# Autodesk Inventor assembly: NewChassis
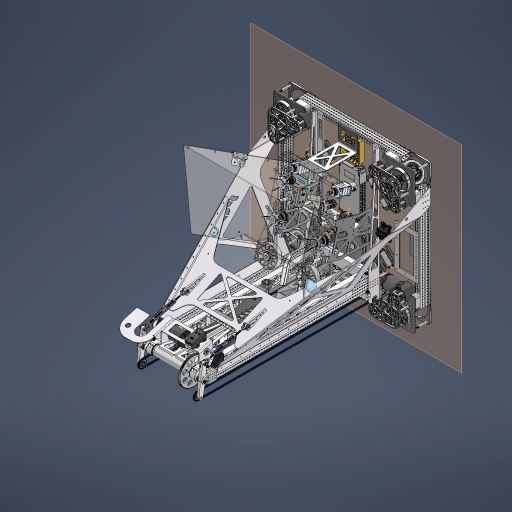
[picture p0: Inventor's stored thumbnail of the model, 512x512]
Saved by Autodesk Inventor 2024.3 (Build 283343000, 343)
## iProperties
ILogicPurgeVersion: 0.0.0.0
OnSaveVersion: 3.5.0.0
OnSaveAssembly: COREAutomationManager
Created: 2025-01-13
Part Number: NewChassis
Document SubType Name: Assembly
Designer: Marcus Tannini
Mfg Approved By: John.Thibert
Mass: 42479.6 g
Surface Area: 120890 cm^2
Volume: 18550.7 cm^3
Density: 2.28991 g/cm^3
ModelCat: Uncategorized
CN_MASS: 42.48
Author: Marcus Tannini
## Documents named in this file (46)
- \\clfs\homes\john.thibert\2025-Poseidon-Mechanical\#Poseidon 2025.iam
- \\clfs\homes\john.thibert\2025-Poseidon-Mechanical\ASSY,MK4i,Swerve_Module_INV.iam
- \\clfs\homes\john.thibert\2025-Poseidon-Mechanical\MAXTube-2x1-Holes.ipt
- \\clfs\homes\john.thibert\2025-Poseidon-Mechanical\BellyPanTop.ipt
- \\clfs\homes\john.thibert\2025-Poseidon-Mechanical\BellyPanBot.ipt
- \\clfs\homes\john.thibert\2025-Poseidon-Mechanical\BATTERY,12V.ipt
- \\clfs\homes\john.thibert\2025-Poseidon-Mechanical\CONTROLS,MAIN_BREAKER.ipt
- \\clfs\homes\john.thibert\2025-Poseidon-Mechanical\CONTROLS,MOTOR,NEO,550.ipt
- \\clfs\homes\john.thibert\2025-Poseidon-Mechanical\CONTROLS,PDH.ipt
- \\clfs\homes\john.thibert\2025-Poseidon-Mechanical\CONTROLS,PH.ipt
- \\clfs\homes\john.thibert\2025-Poseidon-Mechanical\CONTROLS,ROBO_RIO.ipt
- \\clfs\homes\john.thibert\2025-Poseidon-Mechanical\CONTROLS,SPARK_MAX.ipt
- \\clfs\homes\john.thibert\2025-Poseidon-Mechanical\CONTROLS,VRM.ipt
- \\clfs\homes\john.thibert\2025-Poseidon-Mechanical\COVER,SPARKMAX.ipt
- \\clfs\homes\john.thibert\2025-Poseidon-Mechanical\ModifiedCase(IncludesPatterning).iam
- \\clfs\homes\john.thibert\2025-Poseidon-Mechanical\PLATE,MOUNT,BATTERY,TOP.ipt
- \\clfs\homes\john.thibert\2025-Poseidon-Mechanical\SPACER,SPROCKET,IDLER,ELEVATOR.ipt
- \\clfs\homes\john.thibert\2025-Poseidon-Mechanical\PLATE,SIDE,BRACE,RIGHT,ELEVATOR.ipt
- \\clfs\homes\john.thibert\2025-Poseidon-Mechanical\PLATE,SIDE,BRACE,LEFT,ELEVATOR.ipt
- \\clfs\homes\john.thibert\2025-Poseidon-Mechanical\PLATE,TURNBUCKLE,TENSIONER,CHAIN.ipt
- \\clfs\homes\john.thibert\2025-Poseidon-Mechanical\PLATE,BRACE,HORISONTAL,TOP,ELEVATOR.ipt
- \\clfs\homes\john.thibert\2025-Poseidon-Mechanical\TURNBUCKLE,0.25IN_CLEVIS.iam
- \\clfs\homes\john.thibert\2025-Poseidon-Mechanical\STAGE1,ELEVATOR.iam
- \\clfs\homes\john.thibert\2025-Poseidon-Mechanical\ASSY,MAIN,ELEVATOR.iam
- \\clfs\homes\john.thibert\2025-Poseidon-Mechanical\ANGLE,MOUNT,ELEVATOR.ipt
- \\clfs\homes\john.thibert\2025-Poseidon-Mechanical\ANGLE,MOUNT,ELEVATOR,MIRR.ipt
- \\clfs\homes\john.thibert\2025-Poseidon-Mechanical\FABRIC,BUMPERS.ipt
- \\clfs\homes\john.thibert\2025-Poseidon-Mechanical\9293K119_Constant-Force Spring.ipt
- \\clfs\homes\john.thibert\2025-Poseidon-Mechanical\MOUNT,SPRING,ELEVATOR.ipt
- \\clfs\homes\john.thibert\2025-Poseidon-Mechanical\MOUNT,SPRING,ELEVATOR,MIRR.ipt
- \\clfs\homes\john.thibert\2025-Poseidon-Mechanical\SPACER,HEX,0.125IN.ipt
- \\clfs\homes\john.thibert\2025-Poseidon-Mechanical\ARM.iam
- \\clfs\homes\john.thibert\2025-Poseidon-Mechanical\DRIVETRAIN,ELEVATOR.iam
- \\clfs\homes\john.thibert\2025-Poseidon-Mechanical\hopper_assy.iam
- \\clfs\homes\john.thibert\2025-Poseidon-Mechanical\feeder_front_support.ipt
- \\clfs\homes\john.thibert\2025-Poseidon-Mechanical\coral_end_stop.ipt
- \\clfs\homes\john.thibert\2025-Poseidon-Mechanical\coral_end_stop_MIR.ipt
- \\clfs\homes\john.thibert\2025-Poseidon-Mechanical\hopper_backboard.ipt
- \\clfs\homes\john.thibert\2025-Poseidon-Mechanical\Part Studio 1 - Support 1.ipt
- \\clfs\homes\john.thibert\2025-Poseidon-Mechanical\Part Studio 1 - Support 2.ipt
- \\clfs\homes\john.thibert\2025-Poseidon-Mechanical\SDS COLSON.ipt
- \\clfs\homes\john.thibert\2025-Poseidon-Mechanical\SDS LOWERING SPACER.ipt
- \\clfs\homes\john.thibert\2025-Poseidon-Mechanical\#Poseidon 2025\Design Accelerator\Spur Gear21.ipt
- \\clfs\homes\john.thibert\2025-Poseidon-Mechanical\#Poseidon 2025\Design Accelerator\Spur Gear11.ipt
- \\clfs\homes\john.thibert\2025-Poseidon-Mechanical\PLATE,SUPPORT,STOP,ARM.ipt
- \\clfs\homes\john.thibert\2025-Poseidon-Mechanical\PLATE,BRACKET,CABLE_CHAIN.ipt
## Components (81 placed, 47 different names)
1. FABRIC,BUMPERS.ipt:1 — Flush:323, Mate:335, Mate:336
2. Spur Gear1:1 — Mate:708, Mate:709, Flush:325, Rotation:1, Mate:712
3. Spur Gear2:1 — Mate:710, Flush:325, Rotation:1
4. ARM:1 [sub-assembly] — Angle:1, Mate:708, Mate:709, Mate:712, ARM-ANGLE
5. PLATE,BRACKET,CABLE_CHAIN:1 — Flush:326, Mate:722, Mate:723
6. BellyPanBot.ipt:1 — Mate:66, Mate:353, Mate:354
7. BellyPanTop.ipt:1 — Mate:62, Mate:63, Mate:65, Mate:70, Mate:71, Mate:82, Mate:84, Insert:7, Insert:8, Insert:9, Insert:10, Insert:11, Insert:12, Insert:13, Insert:14, Insert:15, Insert:16, Insert:17, Insert:18, Insert:19, Insert:20, Insert:21, Insert:22, Mate:111, Mate:113, Mate:114, Mate:116, Mate:117, Mate:118, Mate:119, Mate:121, Mate:122, Mate:123, Mate:124, Mate:125, Mate:126, Mate:127, Mate:130, Insert:23, Insert:24, Mate:308, Mate:349, Mate:350, Mate:659, Mate:660, Mate:661
8. MAXTube-2x1-Holes.ipt:1 — Mate:3, Mate:4, Mate:115, Mate:272, Mate:687, Mate:692, Mate:696
9. MAXTube-2x1-Holes.ipt:2 — Mate:6, Mate:7, Mate:9, Mate:10, Mate:62, Mate:309, Mate:310
10. MAXTube-2x1-Holes.ipt:3 — Mate:19, Mate:20, Mate:66, Mate:114, Mate:312, Mate:313, Mate:336, Mate:691, Mate:703
11. MAXTube-2x1-Holes.ipt:4 — Mate:12, Mate:13, Mate:16, Mate:17, Mate:29, Mate:63, Mate:271, Mate:353, Mate:354, Mate:678
12. BATTERY,12V.ipt:1 — Mate:356
13. CONTROLS,MAIN_BREAKER.ipt:1 — Mate:82, Mate:111, Mate:116
14. CONTROLS,MOTOR,NEO,550.ipt:1
15. CONTROLS,PDH.ipt:1 — Mate:113, Mate:117, Mate:118, Mate:119
16. CONTROLS,PH.ipt:1 — Insert:23, Insert:24
17. CONTROLS,ROBO_RIO.ipt:1 — Mate:124, Mate:125, Mate:126
18. CONTROLS,SPARK_MAX.ipt:1 — Mate:84, Mate:85, Mate:86, Mate:87
19. CONTROLS,VRM.ipt:1 — Mate:121, Mate:122, Mate:123
20. ModifiedCase(IncludesPatterning).iam:1 [sub-assembly] — Mate:130
21. PLATE,MOUNT,BATTERY,TOP.ipt:1 — Mate:127, Mate:349, Mate:350, Mate:356
22. COVER,SPARKMAX:9 — Mate:724
23. CONTROLS,SPARK_MAX:9 — Mate:655
24. PLATE,SUPPORT,STOP,ARM:1 — Mate:720, Mate:721
25. ASSY,MAIN,ELEVATOR.iam:1 [sub-assembly] — Mate:161, Mate:162, Flush:19, Mate:297, STAGE1 UPPER LIMIT, STAGE1 MAX, Mate:311, Mate:314, Mate:315, Mate:363, Mate:362, Mate:366, Mate:367, Mate:368, Mate:369
26. DRIVETRAIN,ELEVATOR:1 [sub-assembly]
27. STAGE1,ELEVATOR.iam:1 [sub-assembly] — Flush:19, Mate:297, STAGE1 LOWER LIMIT, STAGE1 UPPER LIMIT, STAGE1 DRIVE, STAGE1 MAX, Angle:1, Mate:655, Mate:710, Mate:720, Mate:721, Flush:326, Mate:722, Mate:723, Mate:724, ARM-ANGLE
28. TURNBUCKLE,0.25IN_CLEVIS.iam:1 [sub-assembly]
29. TURNBUCKLE,0.25IN_CLEVIS.iam:2 [sub-assembly] — Mate:707
30. 9293K119_Constant-Force Spring:1 — Mate:364, Mate:365
31. 9293K119_Constant-Force Spring:2 — Mate:370, Mate:371
32. ANGLE,MOUNT,ELEVATOR,MIRR.ipt:1 — Mate:308, Mate:309, Mate:310, Mate:311, Mate:312, Mate:313, Mate:314, Mate:315, Mate:656, Mate:657, Mate:658
33. ANGLE,MOUNT,ELEVATOR.ipt:1 — Mate:65, Mate:70, Mate:71, Mate:161, Mate:162, STAGE1 LOWER LIMIT, STAGE1 DRIVE
34. MOUNT,SPRING,ELEVATOR,MIRR:1 — Mate:367, Mate:368, Mate:369, Mate:370, Mate:371
35. MOUNT,SPRING,ELEVATOR:1 — Mate:363, Mate:362, Mate:364, Mate:365, Mate:366
36. PLATE,BRACE,HORISONTAL,TOP,ELEVATOR.ipt:1 — Mate:285, Mate:286, Mate:289, Mate:290, Mate:291, Mate:295, Mate:296, Mate:668, Mate:669, Mate:670
37. PLATE,SIDE,BRACE,LEFT,ELEVATOR.ipt:1 — Mate:271, Mate:289, Mate:290, Mate:291, Mate:335
38. PLATE,SIDE,BRACE,RIGHT,ELEVATOR.ipt:1 — Mate:272
39. PLATE,TURNBUCKLE,TENSIONER,CHAIN.ipt:1 — Mate:285, Mate:296
40. PLATE,TURNBUCKLE,TENSIONER,CHAIN.ipt:2 — Mate:286, Mate:295, Mate:707
41. SPACER,HEX,0.125IN:1
42. SPACER,SPROCKET,IDLER,ELEVATOR.ipt:1
43. SPACER,SPROCKET,IDLER,ELEVATOR.ipt:2
44. SDS COLSON:1 — Insert:52
45. SDS COLSON:2 — Insert:49
46. SDS COLSON:3 — Insert:50
47. SDS COLSON:4 — Insert:51
48. SDS LOWERING SPACER:1 — Mate:677, Mate:678, Mate:679, Mate:680
49. SDS LOWERING SPACER:2 — Mate:681, Mate:682, Mate:683
50. SDS LOWERING SPACER:3 — Mate:688, Mate:689, Mate:690
51. SDS LOWERING SPACER:4 — Mate:684, Mate:685, Mate:686, Mate:687
52. SDS LOWERING SPACER:5 — Mate:693, Mate:694, Mate:695, Mate:696
53. SDS LOWERING SPACER:6 — Mate:697, Mate:698, Mate:699
54. SDS LOWERING SPACER:7 — Mate:700, Mate:701, Mate:702, Mate:703
55. SDS LOWERING SPACER:8 — Mate:704, Mate:705, Mate:706
56. ASSY,MK4i,Swerve_Module_INV.iam:1 [sub-assembly] — Insert:50, Mate:691, Mate:692, Mate:693, Mate:694, Mate:695, Mate:697, Mate:698, Mate:699
57. ASSY,MK4i,Swerve_Module_INV.iam:2 [sub-assembly] — Mate:3, Mate:4, Mate:6, Mate:7, Insert:51, Mate:684, Mate:685, Mate:686, Mate:688, Mate:689, Mate:690
58. ASSY,MK4i,Swerve_Module_INV.iam:3 [sub-assembly] — Mate:9, Mate:10, Mate:12, Mate:13, Insert:52, Mate:677, Mate:679, Mate:680, Mate:681, Mate:682, Mate:683
59. ASSY,MK4i,Swerve_Module_INV.iam:4 [sub-assembly] — Mate:16, Mate:17, Mate:19, Mate:20, Mate:67, Insert:49, Mate:700, Mate:701, Mate:702, Mate:704, Mate:705, Mate:706
60. CONTROLS,SPARK_MAX.ipt:2
61. CONTROLS,SPARK_MAX.ipt:3
62. CONTROLS,SPARK_MAX.ipt:4
63. CONTROLS,SPARK_MAX.ipt:5
64. CONTROLS,SPARK_MAX.ipt:6
65. CONTROLS,SPARK_MAX.ipt:7
66. CONTROLS,SPARK_MAX.ipt:8
67. COVER,SPARKMAX.ipt:1 — Mate:85, Mate:86, Mate:87, Insert:7, Insert:8
68. COVER,SPARKMAX.ipt:2 — Insert:9, Insert:10
69. COVER,SPARKMAX.ipt:3 — Insert:11, Insert:12
70. COVER,SPARKMAX.ipt:4 — Insert:13, Insert:14
71. COVER,SPARKMAX.ipt:5 — Insert:17, Insert:18
72. COVER,SPARKMAX.ipt:6 — Insert:15, Insert:16
73. COVER,SPARKMAX.ipt:7 — Insert:21, Insert:22
74. COVER,SPARKMAX.ipt:8 — Insert:19, Insert:20
75. hopper_assy:1 [sub-assembly] — Mate:656, Mate:657, Mate:658, Mate:671, Mate:672, Mate:673, Mate:674, Mate:675, Mate:676
76. feeder_front_support:1 — Mate:659, Mate:660, Mate:661, Mate:662, Mate:663, Mate:664, Mate:665, Mate:666, Mate:667
77. coral_end_stop:1 — Mate:665, Mate:666, Mate:667
78. coral_end_stop_MIR:1 — Mate:662, Mate:663, Mate:664
79. hopper_backboard:1 — Mate:668, Mate:669, Mate:670
80. Part Studio 1 - Support 1:1 — Mate:674, Mate:675, Mate:676
81. Part Studio 1 - Support 2:1 — Mate:671, Mate:672, Mate:673
## Relationships (229: Mate 193, Insert 26, Flush 7, Angle 2, RelateRotation 1)
- Mate:3: MAXTube-2x1-Holes.ipt:1 ↔ ASSY,MK4i,Swerve_Module_INV.iam:2
- Mate:4: MAXTube-2x1-Holes.ipt:1 ↔ ASSY,MK4i,Swerve_Module_INV.iam:2
- Mate:6: MAXTube-2x1-Holes.ipt:2 ↔ ASSY,MK4i,Swerve_Module_INV.iam:2
- Mate:7: MAXTube-2x1-Holes.ipt:2 ↔ ASSY,MK4i,Swerve_Module_INV.iam:2
- Mate:9: MAXTube-2x1-Holes.ipt:2 ↔ ASSY,MK4i,Swerve_Module_INV.iam:3
- Mate:10: MAXTube-2x1-Holes.ipt:2 ↔ ASSY,MK4i,Swerve_Module_INV.iam:3
- Mate:12: MAXTube-2x1-Holes.ipt:4 ↔ ASSY,MK4i,Swerve_Module_INV.iam:3
- Mate:13: MAXTube-2x1-Holes.ipt:4 ↔ ASSY,MK4i,Swerve_Module_INV.iam:3
- Mate:16: MAXTube-2x1-Holes.ipt:4 ↔ ASSY,MK4i,Swerve_Module_INV.iam:4
- Mate:17: MAXTube-2x1-Holes.ipt:4 ↔ ASSY,MK4i,Swerve_Module_INV.iam:4
- Mate:19: MAXTube-2x1-Holes.ipt:3 ↔ ASSY,MK4i,Swerve_Module_INV.iam:4
- Mate:20: MAXTube-2x1-Holes.ipt:3 ↔ ASSY,MK4i,Swerve_Module_INV.iam:4
- Mate:29 (-6.35 mm): MAXTube-2x1-Holes.ipt:4
- Mate:62: BellyPanTop.ipt:1 ↔ MAXTube-2x1-Holes.ipt:2
- Mate:63: BellyPanTop.ipt:1 ↔ MAXTube-2x1-Holes.ipt:4
- Mate:65: BellyPanTop.ipt:1 ↔ ANGLE,MOUNT,ELEVATOR.ipt:1
- Mate:66: BellyPanBot.ipt:1 ↔ MAXTube-2x1-Holes.ipt:3
- Mate:67 (35.56 mm): ASSY,MK4i,Swerve_Module_INV.iam:4
- Mate:70: BellyPanTop.ipt:1 ↔ ANGLE,MOUNT,ELEVATOR.ipt:1
- Mate:71: BellyPanTop.ipt:1 ↔ ANGLE,MOUNT,ELEVATOR.ipt:1
- Mate:82: BellyPanTop.ipt:1 ↔ CONTROLS,MAIN_BREAKER.ipt:1
- Mate:84: BellyPanTop.ipt:1 ↔ CONTROLS,SPARK_MAX.ipt:1
- Mate:85: CONTROLS,SPARK_MAX.ipt:1 ↔ COVER,SPARKMAX.ipt:1
- Mate:86: CONTROLS,SPARK_MAX.ipt:1 ↔ COVER,SPARKMAX.ipt:1
- Mate:87: CONTROLS,SPARK_MAX.ipt:1 ↔ COVER,SPARKMAX.ipt:1
- Insert:7: BellyPanTop.ipt:1 ↔ COVER,SPARKMAX.ipt:1
- Insert:8: BellyPanTop.ipt:1 ↔ COVER,SPARKMAX.ipt:1
- [Mate]: CONTROLS,SPARK_MAX.ipt:2 ↔ COVER,SPARKMAX.ipt:2
- [Mate]: CONTROLS,SPARK_MAX.ipt:2 ↔ COVER,SPARKMAX.ipt:2
- [Mate]: CONTROLS,SPARK_MAX.ipt:2 ↔ COVER,SPARKMAX.ipt:2
- [Mate]: CONTROLS,SPARK_MAX.ipt:3 ↔ COVER,SPARKMAX.ipt:3
- [Mate]: CONTROLS,SPARK_MAX.ipt:3 ↔ COVER,SPARKMAX.ipt:3
- [Mate]: CONTROLS,SPARK_MAX.ipt:3 ↔ COVER,SPARKMAX.ipt:3
- [Mate]: CONTROLS,SPARK_MAX.ipt:4 ↔ COVER,SPARKMAX.ipt:4
- [Mate]: CONTROLS,SPARK_MAX.ipt:4 ↔ COVER,SPARKMAX.ipt:4
- [Mate]: CONTROLS,SPARK_MAX.ipt:4 ↔ COVER,SPARKMAX.ipt:4
- [Mate]: CONTROLS,SPARK_MAX.ipt:5 ↔ COVER,SPARKMAX.ipt:5
- [Mate]: CONTROLS,SPARK_MAX.ipt:5 ↔ COVER,SPARKMAX.ipt:5
- [Mate]: CONTROLS,SPARK_MAX.ipt:5 ↔ COVER,SPARKMAX.ipt:5
- [Mate]: CONTROLS,SPARK_MAX.ipt:6 ↔ COVER,SPARKMAX.ipt:6
- [Mate]: CONTROLS,SPARK_MAX.ipt:6 ↔ COVER,SPARKMAX.ipt:6
- [Mate]: CONTROLS,SPARK_MAX.ipt:6 ↔ COVER,SPARKMAX.ipt:6
- [Mate]: CONTROLS,SPARK_MAX.ipt:7 ↔ COVER,SPARKMAX.ipt:7
- [Mate]: CONTROLS,SPARK_MAX.ipt:7 ↔ COVER,SPARKMAX.ipt:7
- [Mate]: CONTROLS,SPARK_MAX.ipt:7 ↔ COVER,SPARKMAX.ipt:7
- [Mate]: CONTROLS,SPARK_MAX.ipt:8 ↔ COVER,SPARKMAX.ipt:8
- [Mate]: CONTROLS,SPARK_MAX.ipt:8 ↔ COVER,SPARKMAX.ipt:8
- [Mate]: CONTROLS,SPARK_MAX.ipt:8 ↔ COVER,SPARKMAX.ipt:8
- Insert:9: BellyPanTop.ipt:1 ↔ COVER,SPARKMAX.ipt:2
- Insert:10: BellyPanTop.ipt:1 ↔ COVER,SPARKMAX.ipt:2
- Insert:11: BellyPanTop.ipt:1 ↔ COVER,SPARKMAX.ipt:3
- Insert:12: BellyPanTop.ipt:1 ↔ COVER,SPARKMAX.ipt:3
- Insert:13: BellyPanTop.ipt:1 ↔ COVER,SPARKMAX.ipt:4
- Insert:14: BellyPanTop.ipt:1 ↔ COVER,SPARKMAX.ipt:4
- Insert:15: BellyPanTop.ipt:1 ↔ COVER,SPARKMAX.ipt:6
- Insert:16: BellyPanTop.ipt:1 ↔ COVER,SPARKMAX.ipt:6
- Insert:17: BellyPanTop.ipt:1 ↔ COVER,SPARKMAX.ipt:5
- Insert:18: BellyPanTop.ipt:1 ↔ COVER,SPARKMAX.ipt:5
- Insert:19: BellyPanTop.ipt:1 ↔ COVER,SPARKMAX.ipt:8
- Insert:20: BellyPanTop.ipt:1 ↔ COVER,SPARKMAX.ipt:8
- Insert:21: BellyPanTop.ipt:1 ↔ COVER,SPARKMAX.ipt:7
- Insert:22: BellyPanTop.ipt:1 ↔ COVER,SPARKMAX.ipt:7
- Mate:111: BellyPanTop.ipt:1 ↔ CONTROLS,MAIN_BREAKER.ipt:1
- Mate:113: BellyPanTop.ipt:1 ↔ CONTROLS,PDH.ipt:1
- Mate:114: BellyPanTop.ipt:1 ↔ MAXTube-2x1-Holes.ipt:3
- Mate:115 (-374.65 mm): MAXTube-2x1-Holes.ipt:1
- Mate:116 (0.254 mm): BellyPanTop.ipt:1 ↔ CONTROLS,MAIN_BREAKER.ipt:1
- Mate:117: BellyPanTop.ipt:1 ↔ CONTROLS,PDH.ipt:1
- Mate:118: BellyPanTop.ipt:1 ↔ CONTROLS,PDH.ipt:1
- Mate:119: BellyPanTop.ipt:1 ↔ CONTROLS,PDH.ipt:1
- Mate:121: BellyPanTop.ipt:1 ↔ CONTROLS,VRM.ipt:1
- Mate:122: BellyPanTop.ipt:1 ↔ CONTROLS,VRM.ipt:1
- Mate:123: BellyPanTop.ipt:1 ↔ CONTROLS,VRM.ipt:1
- Mate:124: BellyPanTop.ipt:1 ↔ CONTROLS,ROBO_RIO.ipt:1
- Mate:125: BellyPanTop.ipt:1 ↔ CONTROLS,ROBO_RIO.ipt:1
- Mate:126: BellyPanTop.ipt:1 ↔ CONTROLS,ROBO_RIO.ipt:1
- Mate:127: BellyPanTop.ipt:1 ↔ PLATE,MOUNT,BATTERY,TOP.ipt:1
- Mate:130: BellyPanTop.ipt:1 ↔ ModifiedCase(IncludesPatterning).iam:1
- Insert:23: BellyPanTop.ipt:1 ↔ CONTROLS,PH.ipt:1
- Insert:24: BellyPanTop.ipt:1 ↔ CONTROLS,PH.ipt:1
- Mate:161: ASSY,MAIN,ELEVATOR.iam:1 ↔ ANGLE,MOUNT,ELEVATOR.ipt:1
- Mate:162: ASSY,MAIN,ELEVATOR.iam:1 ↔ ANGLE,MOUNT,ELEVATOR.ipt:1
- [Mate]: ASSY,MAIN,ELEVATOR.iam:1 ↔ ANGLE,MOUNT,ELEVATOR.ipt:1
- [Insert]: ASSY,MAIN,ELEVATOR.iam:1 ↔ SPACER,SPROCKET,IDLER,ELEVATOR.ipt:1
- [Insert]: ASSY,MAIN,ELEVATOR.iam:1 ↔ SPACER,SPROCKET,IDLER,ELEVATOR.ipt:1
- [Flush]: ASSY,MAIN,ELEVATOR.iam:1 ↔ DRIVETRAIN,ELEVATOR:1
- [Insert]: ASSY,MAIN,ELEVATOR.iam:1 ↔ SPACER,SPROCKET,IDLER,ELEVATOR.ipt:2
- [Insert]: ASSY,MAIN,ELEVATOR.iam:1 ↔ SPACER,SPROCKET,IDLER,ELEVATOR.ipt:2
- [Mate]: BellyPanTop.ipt:1 ↔ DRIVETRAIN,ELEVATOR:1
- [Mate]: DRIVETRAIN,ELEVATOR:1 ↔ ANGLE,MOUNT,ELEVATOR.ipt:1
- [Flush]: ASSY,MAIN,ELEVATOR.iam:1 ↔ DRIVETRAIN,ELEVATOR:1
- [Mate]: ASSY,MAIN,ELEVATOR.iam:1 ↔ PLATE,SIDE,BRACE,LEFT,ELEVATOR.ipt:1
- [Mate]: ASSY,MAIN,ELEVATOR.iam:1 ↔ PLATE,SIDE,BRACE,LEFT,ELEVATOR.ipt:1
- [Mate]: ASSY,MAIN,ELEVATOR.iam:1 ↔ DRIVETRAIN,ELEVATOR:1
- [Mate]: ASSY,MAIN,ELEVATOR.iam:1 ↔ PLATE,SIDE,BRACE,LEFT,ELEVATOR.ipt:1
- [Mate]: ASSY,MAIN,ELEVATOR.iam:1 ↔ PLATE,SIDE,BRACE,RIGHT,ELEVATOR.ipt:1
- [Mate]: ASSY,MAIN,ELEVATOR.iam:1 ↔ PLATE,SIDE,BRACE,RIGHT,ELEVATOR.ipt:1
- [Mate]: ASSY,MAIN,ELEVATOR.iam:1 ↔ PLATE,SIDE,BRACE,RIGHT,ELEVATOR.ipt:1
- Mate:271: MAXTube-2x1-Holes.ipt:4 ↔ PLATE,SIDE,BRACE,LEFT,ELEVATOR.ipt:1
- Mate:272: MAXTube-2x1-Holes.ipt:1 ↔ PLATE,SIDE,BRACE,RIGHT,ELEVATOR.ipt:1
- [Mate]: ASSY,MAIN,ELEVATOR.iam:1 ↔ TURNBUCKLE,0.25IN_CLEVIS.iam:1
- [Mate]: ASSY,MAIN,ELEVATOR.iam:1 ↔ TURNBUCKLE,0.25IN_CLEVIS.iam:1
- [Mate]: ASSY,MAIN,ELEVATOR.iam:1 ↔ TURNBUCKLE,0.25IN_CLEVIS.iam:2
- [Mate]: ASSY,MAIN,ELEVATOR.iam:1 ↔ TURNBUCKLE,0.25IN_CLEVIS.iam:2
- Mate:285: PLATE,BRACE,HORISONTAL,TOP,ELEVATOR.ipt:1 ↔ PLATE,TURNBUCKLE,TENSIONER,CHAIN.ipt:1
- Mate:286: PLATE,BRACE,HORISONTAL,TOP,ELEVATOR.ipt:1 ↔ PLATE,TURNBUCKLE,TENSIONER,CHAIN.ipt:2
- Mate:289: PLATE,BRACE,HORISONTAL,TOP,ELEVATOR.ipt:1 ↔ PLATE,SIDE,BRACE,LEFT,ELEVATOR.ipt:1
- Mate:290: PLATE,BRACE,HORISONTAL,TOP,ELEVATOR.ipt:1 ↔ PLATE,SIDE,BRACE,LEFT,ELEVATOR.ipt:1
- Mate:291: PLATE,BRACE,HORISONTAL,TOP,ELEVATOR.ipt:1 ↔ PLATE,SIDE,BRACE,LEFT,ELEVATOR.ipt:1
- [Mate]: ASSY,MAIN,ELEVATOR.iam:1 ↔ DRIVETRAIN,ELEVATOR:1
- Mate:295: PLATE,BRACE,HORISONTAL,TOP,ELEVATOR.ipt:1 ↔ PLATE,TURNBUCKLE,TENSIONER,CHAIN.ipt:2
- Mate:296: PLATE,BRACE,HORISONTAL,TOP,ELEVATOR.ipt:1 ↔ PLATE,TURNBUCKLE,TENSIONER,CHAIN.ipt:1
- Flush:19: ASSY,MAIN,ELEVATOR.iam:1 ↔ STAGE1,ELEVATOR.iam:1
- Mate:297: ASSY,MAIN,ELEVATOR.iam:1 ↔ STAGE1,ELEVATOR.iam:1
- STAGE1 LOWER LIMIT [Mate]: STAGE1,ELEVATOR.iam:1 ↔ ANGLE,MOUNT,ELEVATOR.ipt:1
- STAGE1 UPPER LIMIT [Mate]: ASSY,MAIN,ELEVATOR.iam:1 ↔ STAGE1,ELEVATOR.iam:1
- STAGE1 DRIVE [Mate]: STAGE1,ELEVATOR.iam:1 ↔ ANGLE,MOUNT,ELEVATOR.ipt:1
- STAGE1 MAX [Mate] (3.175 mm): ASSY,MAIN,ELEVATOR.iam:1 ↔ STAGE1,ELEVATOR.iam:1
- Mate:308: BellyPanTop.ipt:1 ↔ ANGLE,MOUNT,ELEVATOR,MIRR.ipt:1
- Mate:309: MAXTube-2x1-Holes.ipt:2 ↔ ANGLE,MOUNT,ELEVATOR,MIRR.ipt:1
- Mate:310: MAXTube-2x1-Holes.ipt:2 ↔ ANGLE,MOUNT,ELEVATOR,MIRR.ipt:1
- Mate:311: ASSY,MAIN,ELEVATOR.iam:1 ↔ ANGLE,MOUNT,ELEVATOR,MIRR.ipt:1
- Mate:312: MAXTube-2x1-Holes.ipt:3 ↔ ANGLE,MOUNT,ELEVATOR,MIRR.ipt:1
- Mate:313: MAXTube-2x1-Holes.ipt:3 ↔ ANGLE,MOUNT,ELEVATOR,MIRR.ipt:1
- Mate:314: ASSY,MAIN,ELEVATOR.iam:1 ↔ ANGLE,MOUNT,ELEVATOR,MIRR.ipt:1
- Mate:315: ASSY,MAIN,ELEVATOR.iam:1 ↔ ANGLE,MOUNT,ELEVATOR,MIRR.ipt:1
- Flush:323 (146.05 mm): FABRIC,BUMPERS.ipt:1
- Mate:335 (3.175 mm): FABRIC,BUMPERS.ipt:1 ↔ PLATE,SIDE,BRACE,LEFT,ELEVATOR.ipt:1
- Mate:336 (6.35 mm): FABRIC,BUMPERS.ipt:1 ↔ MAXTube-2x1-Holes.ipt:3
- Mate:349: BellyPanTop.ipt:1 ↔ PLATE,MOUNT,BATTERY,TOP.ipt:1
- Mate:350: BellyPanTop.ipt:1 ↔ PLATE,MOUNT,BATTERY,TOP.ipt:1
- Mate:353: BellyPanBot.ipt:1 ↔ MAXTube-2x1-Holes.ipt:4
- Mate:354: BellyPanBot.ipt:1 ↔ MAXTube-2x1-Holes.ipt:4
- Mate:356 (19.05 mm): BATTERY,12V.ipt:1 ↔ PLATE,MOUNT,BATTERY,TOP.ipt:1
- Mate:363: ASSY,MAIN,ELEVATOR.iam:1 ↔ MOUNT,SPRING,ELEVATOR:1
- Mate:362: ASSY,MAIN,ELEVATOR.iam:1 ↔ MOUNT,SPRING,ELEVATOR:1
- Mate:364: 9293K119_Constant-Force Spring:1 ↔ MOUNT,SPRING,ELEVATOR:1
- Mate:365 (1.5875 mm): 9293K119_Constant-Force Spring:1 ↔ MOUNT,SPRING,ELEVATOR:1
- Mate:366: ASSY,MAIN,ELEVATOR.iam:1 ↔ MOUNT,SPRING,ELEVATOR:1
- Mate:367: ASSY,MAIN,ELEVATOR.iam:1 ↔ MOUNT,SPRING,ELEVATOR,MIRR:1
- Mate:368: ASSY,MAIN,ELEVATOR.iam:1 ↔ MOUNT,SPRING,ELEVATOR,MIRR:1
- Mate:369: ASSY,MAIN,ELEVATOR.iam:1 ↔ MOUNT,SPRING,ELEVATOR,MIRR:1
- Mate:370: 9293K119_Constant-Force Spring:2 ↔ MOUNT,SPRING,ELEVATOR,MIRR:1
- Mate:371 (1.5875 mm): 9293K119_Constant-Force Spring:2 ↔ MOUNT,SPRING,ELEVATOR,MIRR:1
- [Mate] (0.254 mm): ASSY,MAIN,ELEVATOR.iam:1 ↔ DRIVETRAIN,ELEVATOR:1
- [Mate]: ASSY,MAIN,ELEVATOR.iam:1 ↔ DRIVETRAIN,ELEVATOR:1
- [Mate]: DRIVETRAIN,ELEVATOR:1 ↔ SPACER,HEX,0.125IN:1
- [Mate]: DRIVETRAIN,ELEVATOR:1 ↔ SPACER,HEX,0.125IN:1
- [Mate]: ARM:1 ↔ STAGE1,ELEVATOR.iam:1
- [Mate]: ARM:1 ↔ STAGE1,ELEVATOR.iam:1
- [Mate]: MAXTube-2x1-Holes.ipt:2 ↔ DRIVETRAIN,ELEVATOR:1
- [Mate]: MAXTube-2x1-Holes.ipt:2 ↔ DRIVETRAIN,ELEVATOR:1
- [Mate]: ARM:1 ↔ STAGE1,ELEVATOR.iam:1
- [Mate]: ARM:1 ↔ STAGE1,ELEVATOR.iam:1
- Angle:1 (0 deg): ARM:1 ↔ STAGE1,ELEVATOR.iam:1
- [Mate]: COVER,SPARKMAX:9 ↔ CONTROLS,SPARK_MAX:9
- [Mate]: COVER,SPARKMAX:9 ↔ CONTROLS,SPARK_MAX:9
- [Mate]: COVER,SPARKMAX:9 ↔ CONTROLS,SPARK_MAX:9
- Mate:655: CONTROLS,SPARK_MAX:9 ↔ STAGE1,ELEVATOR.iam:1
- Mate:656: ANGLE,MOUNT,ELEVATOR,MIRR.ipt:1 ↔ hopper_assy:1
- Mate:657: ANGLE,MOUNT,ELEVATOR,MIRR.ipt:1 ↔ hopper_assy:1
- Mate:658: ANGLE,MOUNT,ELEVATOR,MIRR.ipt:1 ↔ hopper_assy:1
- Mate:659: BellyPanTop.ipt:1 ↔ feeder_front_support:1
- Mate:660: BellyPanTop.ipt:1 ↔ feeder_front_support:1
- Mate:661: BellyPanTop.ipt:1 ↔ feeder_front_support:1
- Mate:662: feeder_front_support:1 ↔ coral_end_stop_MIR:1
- Mate:663: feeder_front_support:1 ↔ coral_end_stop_MIR:1
- Mate:664: feeder_front_support:1 ↔ coral_end_stop_MIR:1
- Mate:665: feeder_front_support:1 ↔ coral_end_stop:1
- Mate:666: feeder_front_support:1 ↔ coral_end_stop:1
- Mate:667: feeder_front_support:1 ↔ coral_end_stop:1
- Mate:668: PLATE,BRACE,HORISONTAL,TOP,ELEVATOR.ipt:1 ↔ hopper_backboard:1
- Mate:669: PLATE,BRACE,HORISONTAL,TOP,ELEVATOR.ipt:1 ↔ hopper_backboard:1
- Mate:670: PLATE,BRACE,HORISONTAL,TOP,ELEVATOR.ipt:1 ↔ hopper_backboard:1
- Mate:671: hopper_assy:1 ↔ Part Studio 1 - Support 2:1
- Mate:672: hopper_assy:1 ↔ Part Studio 1 - Support 2:1
- Mate:673: hopper_assy:1 ↔ Part Studio 1 - Support 2:1
- Mate:674: hopper_assy:1 ↔ Part Studio 1 - Support 1:1
- Mate:675: hopper_assy:1 ↔ Part Studio 1 - Support 1:1
- Mate:676: hopper_assy:1 ↔ Part Studio 1 - Support 1:1
- Insert:49: SDS COLSON:2 ↔ ASSY,MK4i,Swerve_Module_INV.iam:4
- Insert:50: SDS COLSON:3 ↔ ASSY,MK4i,Swerve_Module_INV.iam:1
- Insert:51: SDS COLSON:4 ↔ ASSY,MK4i,Swerve_Module_INV.iam:2
- Insert:52: SDS COLSON:1 ↔ ASSY,MK4i,Swerve_Module_INV.iam:3
- Mate:677: SDS LOWERING SPACER:1 ↔ ASSY,MK4i,Swerve_Module_INV.iam:3
- Mate:678: MAXTube-2x1-Holes.ipt:4 ↔ SDS LOWERING SPACER:1
- Mate:679: SDS LOWERING SPACER:1 ↔ ASSY,MK4i,Swerve_Module_INV.iam:3
- Mate:680: SDS LOWERING SPACER:1 ↔ ASSY,MK4i,Swerve_Module_INV.iam:3
- Mate:681: SDS LOWERING SPACER:2 ↔ ASSY,MK4i,Swerve_Module_INV.iam:3
- Mate:682: SDS LOWERING SPACER:2 ↔ ASSY,MK4i,Swerve_Module_INV.iam:3
- Mate:683: SDS LOWERING SPACER:2 ↔ ASSY,MK4i,Swerve_Module_INV.iam:3
- Mate:684: SDS LOWERING SPACER:4 ↔ ASSY,MK4i,Swerve_Module_INV.iam:2
- Mate:685: SDS LOWERING SPACER:4 ↔ ASSY,MK4i,Swerve_Module_INV.iam:2
- Mate:686: SDS LOWERING SPACER:4 ↔ ASSY,MK4i,Swerve_Module_INV.iam:2
- Mate:687: MAXTube-2x1-Holes.ipt:1 ↔ SDS LOWERING SPACER:4
- Mate:688: SDS LOWERING SPACER:3 ↔ ASSY,MK4i,Swerve_Module_INV.iam:2
- Mate:689: SDS LOWERING SPACER:3 ↔ ASSY,MK4i,Swerve_Module_INV.iam:2
- Mate:690: SDS LOWERING SPACER:3 ↔ ASSY,MK4i,Swerve_Module_INV.iam:2
- Mate:691: MAXTube-2x1-Holes.ipt:3 ↔ ASSY,MK4i,Swerve_Module_INV.iam:1
- Mate:692: MAXTube-2x1-Holes.ipt:1 ↔ ASSY,MK4i,Swerve_Module_INV.iam:1
- Mate:693: SDS LOWERING SPACER:5 ↔ ASSY,MK4i,Swerve_Module_INV.iam:1
- Mate:694: SDS LOWERING SPACER:5 ↔ ASSY,MK4i,Swerve_Module_INV.iam:1
- Mate:695: SDS LOWERING SPACER:5 ↔ ASSY,MK4i,Swerve_Module_INV.iam:1
- Mate:696: MAXTube-2x1-Holes.ipt:1 ↔ SDS LOWERING SPACER:5
- Mate:697: SDS LOWERING SPACER:6 ↔ ASSY,MK4i,Swerve_Module_INV.iam:1
- Mate:698: SDS LOWERING SPACER:6 ↔ ASSY,MK4i,Swerve_Module_INV.iam:1
- Mate:699: SDS LOWERING SPACER:6 ↔ ASSY,MK4i,Swerve_Module_INV.iam:1
- Mate:700: SDS LOWERING SPACER:7 ↔ ASSY,MK4i,Swerve_Module_INV.iam:4
- Mate:701: SDS LOWERING SPACER:7 ↔ ASSY,MK4i,Swerve_Module_INV.iam:4
- Mate:702: SDS LOWERING SPACER:7 ↔ ASSY,MK4i,Swerve_Module_INV.iam:4
- Mate:703: MAXTube-2x1-Holes.ipt:3 ↔ SDS LOWERING SPACER:7
- Mate:704: SDS LOWERING SPACER:8 ↔ ASSY,MK4i,Swerve_Module_INV.iam:4
- Mate:705: SDS LOWERING SPACER:8 ↔ ASSY,MK4i,Swerve_Module_INV.iam:4
- Mate:706: SDS LOWERING SPACER:8 ↔ ASSY,MK4i,Swerve_Module_INV.iam:4
- Mate:707: TURNBUCKLE,0.25IN_CLEVIS.iam:2 ↔ PLATE,TURNBUCKLE,TENSIONER,CHAIN.ipt:2
- Flush:324 (25.75 mm)
- Mate:708: Spur Gear1:1 ↔ ARM:1
- Mate:709: Spur Gear1:1 ↔ ARM:1
- Mate:710: Spur Gear2:1 ↔ STAGE1,ELEVATOR.iam:1
- Flush:325: Spur Gear1:1 ↔ Spur Gear2:1
- Rotation:1 [RelateRotation] (4 ul): Spur Gear1:1 ↔ Spur Gear2:1
- Mate:712: Spur Gear1:1 ↔ ARM:1
- Mate:720: PLATE,SUPPORT,STOP,ARM:1 ↔ STAGE1,ELEVATOR.iam:1
- Mate:721: PLATE,SUPPORT,STOP,ARM:1 ↔ STAGE1,ELEVATOR.iam:1
- Flush:326: PLATE,BRACKET,CABLE_CHAIN:1 ↔ STAGE1,ELEVATOR.iam:1
- Mate:722: PLATE,BRACKET,CABLE_CHAIN:1 ↔ STAGE1,ELEVATOR.iam:1
- Mate:723: PLATE,BRACKET,CABLE_CHAIN:1 ↔ STAGE1,ELEVATOR.iam:1
- Mate:724: COVER,SPARKMAX:9 ↔ STAGE1,ELEVATOR.iam:1
- ARM-ANGLE [Angle] (90 deg): ARM:1 ↔ STAGE1,ELEVATOR.iam:1
## Named parameters: d160_d155 = 0 mm, d161_d156 = 0 mm, d162_d157 = 0 mm, d163_d155 = 0 mm, d164_d156 = 0 mm, d165_d157 = 0 mm, d166_d155 = 0 mm, d167_d156 = 0 mm, d168_d157 = 0 mm, d169_d155 = 0 mm, d170_d156 = 0 mm, d171_d157 = 0 mm, d172_d155 = 0 mm, d173_d156 = 0 mm, d174_d157 = 0 mm, d175_d155 = 0 mm, d176_d156 = 0 mm, d177_d157 = 0 mm, d178_d155 = 0 mm, d179_d156 = 0 mm, d180_d157 = 0 mm, d518_d513 = 0 mm, d1392_d178_d155 = 0 mm, d1393_d179_d156 = 0 mm, d1394_d180_d157 = 0 mm
